# Autodesk Inventor assembly: 組合2
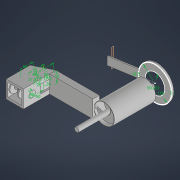
[picture p0: Inventor's stored thumbnail of the model, 180x180]
Saved by Autodesk Inventor 2021 (Build 250183000, 183)
## iProperties
Created: 2020-12-30
Part Number: 組合2
Document SubType Name: Assembly
Designer: zihon
Author: zihon
## Documents named in this file (10)
- C:\Users\zihon\Desktop\New folder\組合2.iam
- C:\Users\zihon\Desktop\New folder\架.ipt
- C:\Users\zihon\Desktop\New folder\零件1.ipt
- C:\Users\zihon\Desktop\New folder\零件2.ipt
- C:\Users\zihon\Desktop\New folder\零件3.ipt
- C:\Users\zihon\Desktop\New folder\零件4.ipt
- C:\Users\zihon\Desktop\New folder\軸.ipt
- C:\Users\zihon\Desktop\New folder\直線軌道.ipt
- C:\Users\zihon\Desktop\New folder\螺旋.ipt
- C:\Users\zihon\Desktop\New folder\盤.ipt
## Components (9 placed, 9 different names)
1. 架:1 — 貼合:1, 貼合:2, 齊平:1, 貼合:4, 貼合:6, 貼合:8, 貼合:9, 貼合:11, 齊平:2, 貼合:13, 貼合:14, 貼合:15, 貼合:16, 貼合:17, 貼合:18
2. 零件1:1 — 貼合:4, 相切:1, 貼合:18
3. 零件2:1 — 貼合:6, 相切:2, 貼合:17
4. 零件3:1 — 貼合:8, 相切:3, 貼合:16
5. 零件4:1 — 貼合:9, 相切:4, 貼合:15
6. 軸:1 — 貼合:11, 齊平:2, 相切:1, 相切:2, 相切:3, 相切:4
7. 直線軌道:1 — 齊平:3, 貼合:13, 貼合:14, 貼合:21
8. 螺旋:1 — 貼合:19, 貼合:20, 貼合:21
9. 盤:1
## Relationships (23: Mate 16, Tangent 4, Flush 3)
- 貼合:1 [Mate]: 架:1
- 貼合:2 [Mate]: 架:1
- 齊平:1 [Flush]: 架:1
- 貼合:4 [Mate]: 架:1 ↔ 零件1:1
- 貼合:6 [Mate]: 架:1 ↔ 零件2:1
- 貼合:8 [Mate]: 架:1 ↔ 零件3:1
- 貼合:9 [Mate]: 架:1 ↔ 零件4:1
- 貼合:11 [Mate]: 架:1 ↔ 軸:1
- 齊平:2 [Flush]: 架:1 ↔ 軸:1
- 相切:1 [Tangent]: 零件1:1 ↔ 軸:1
- 相切:2 [Tangent]: 零件2:1 ↔ 軸:1
- 相切:3 [Tangent]: 零件3:1 ↔ 軸:1
- 相切:4 [Tangent]: 零件4:1 ↔ 軸:1
- 齊平:3 [Flush]: 直線軌道:1
- 貼合:13 [Mate]: 架:1 ↔ 直線軌道:1
- 貼合:14 [Mate]: 架:1 ↔ 直線軌道:1
- 貼合:15 [Mate]: 架:1 ↔ 零件4:1
- 貼合:16 [Mate]: 架:1 ↔ 零件3:1
- 貼合:17 [Mate]: 架:1 ↔ 零件2:1
- 貼合:18 [Mate]: 架:1 ↔ 零件1:1
- 貼合:19 [Mate]: 螺旋:1
- 貼合:20 [Mate]: 螺旋:1
- 貼合:21 [Mate] (45.101 mm): 直線軌道:1 ↔ 螺旋:1
